# Autodesk Inventor assembly: Front Hub Carrier L
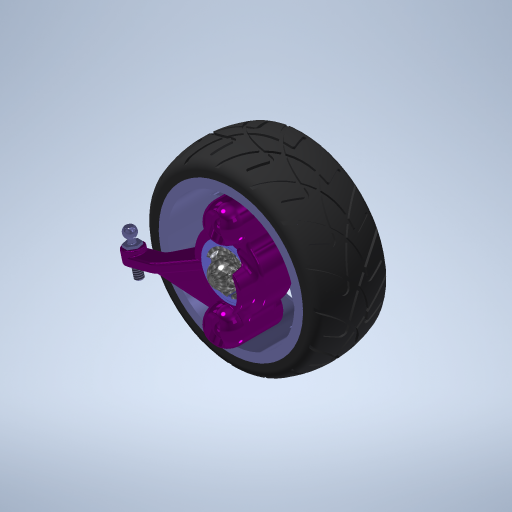
[picture p0: Inventor's stored thumbnail of the model, 512x512]
Saved by Autodesk Inventor 2023.1 (Build 271208000, 208)
## iProperties
Created: 2019-12-03
Part Number: Front Hub Carrier L
Document SubType Name: Assembly
Designer: Jopa
Author: Jopa
## Documents named in this file (13)
- C:\Users\Arzum Naz Doğaner\OneDrive\Masaüstü\HUDSON süspansiyon\Front Hub Carrier L.iam
- C:\Users\Arzum Naz Doğaner\OneDrive\Masaüstü\HUDSON süspansiyon\Front Hub Carrier L.ipt
- C:\Users\Arzum Naz Doğaner\OneDrive\Masaüstü\HUDSON süspansiyon\Pillow Ball Retainer.ipt
- C:\Users\Arzum Naz Doğaner\OneDrive\Masaüstü\HUDSON süspansiyon\Pillow Ball Bushing.ipt
- C:\Users\Jopa\Desktop\Suspension\Pillow Ball Retainer_CPY.ipt
- C:\Users\Jopa\Desktop\Suspension\Pillow Ball Bushing_CPY.ipt
- C:\Users\Arzum Naz Doğaner\OneDrive\Masaüstü\HUDSON süspansiyon\Rear Hub Bearing.ipt
- C:\Users\Arzum Naz Doğaner\OneDrive\Masaüstü\HUDSON süspansiyon\Front Axel.ipt
- C:\Users\Arzum Naz Doğaner\OneDrive\Masaüstü\HUDSON süspansiyon\Front Hub Bearing.ipt
- C:\Users\Arzum Naz Doğaner\OneDrive\Masaüstü\HUDSON süspansiyon\0.1875 Ball Stud 0.375.ipt
- C:\Users\Arzum Naz Doğaner\OneDrive\Masaüstü\HUDSON süspansiyon\Rear Hex Hub.iam
- C:\Users\Arzum Naz Doğaner\OneDrive\Masaüstü\HUDSON süspansiyon\Wheel L.iam
- C:\Users\Arzum Naz Doğaner\OneDrive\Masaüstü\HUDSON süspansiyon\ANSI B18.2.4.4M - M5 x 0,8.ipt
## Components (12 placed, 12 different names)
1. Front Hub Carrier L:1 — Mate:3, Mate:4, Mate:7, Mate:8, Insert:1, Mate:9, Insert:2, Insert:3
2. Pillow Ball Retainer:1 — Mate:1, Mate:2, Mate:3
3. Pillow Ball Bushing:1 — Mate:1, Mate:2, Mate:4
4. Pillow Ball Retainer_CPY:1 — Mate:5, Mate:6, Mate:8
5. Pillow Ball Bushing_CPY:1 — Mate:5, Mate:6, Mate:7
6. Rear Hub Bearing:1 — Insert:1
7. Front Axel:1 — Mate:9, Mate:10, Mate:11, Mate:12, Mate:13, Mate:16
8. Front Hub Bearing:1 — Insert:2, Mate:10
9. 0.1875 Ball Stud 0.375:1 — Insert:3
10. Rear Hex Hub:1 [sub-assembly] — Mate:11, Mate:12, Mate:14, Mate:15
11. Wheel L:1 [sub-assembly] — Mate:13, Mate:14, Mate:15, Mate:17
12. ANSI B18.2.4.4M - M5 x 0,8:1 — Mate:16, Mate:17
## Relationships (20: Mate 17, Insert 3)
- Mate:1: Pillow Ball Retainer:1 ↔ Pillow Ball Bushing:1
- Mate:2: Pillow Ball Retainer:1 ↔ Pillow Ball Bushing:1
- Mate:3: Front Hub Carrier L:1 ↔ Pillow Ball Retainer:1
- Mate:4: Front Hub Carrier L:1 ↔ Pillow Ball Bushing:1
- Mate:5: Pillow Ball Retainer_CPY:1 ↔ Pillow Ball Bushing_CPY:1
- Mate:6: Pillow Ball Retainer_CPY:1 ↔ Pillow Ball Bushing_CPY:1
- Mate:7: Front Hub Carrier L:1 ↔ Pillow Ball Bushing_CPY:1
- Mate:8: Front Hub Carrier L:1 ↔ Pillow Ball Retainer_CPY:1
- Insert:1: Front Hub Carrier L:1 ↔ Rear Hub Bearing:1
- Mate:9: Front Hub Carrier L:1 ↔ Front Axel:1
- Insert:2: Front Hub Carrier L:1 ↔ Front Hub Bearing:1
- Mate:10: Front Axel:1 ↔ Front Hub Bearing:1
- Insert:3: Front Hub Carrier L:1 ↔ 0.1875 Ball Stud 0.375:1
- Mate:11: Front Axel:1 ↔ Rear Hex Hub:1
- Mate:12: Front Axel:1 ↔ Rear Hex Hub:1
- Mate:13: Front Axel:1 ↔ Wheel L:1
- Mate:14: Rear Hex Hub:1 ↔ Wheel L:1
- Mate:15: Rear Hex Hub:1 ↔ Wheel L:1
- Mate:16: Front Axel:1 ↔ ANSI B18.2.4.4M - M5 x 0,8:1
- Mate:17: Wheel L:1 ↔ ANSI B18.2.4.4M - M5 x 0,8:1
